# Autodesk Inventor assembly: 200-02-ROCKER-CONNECTOR-ASM-L
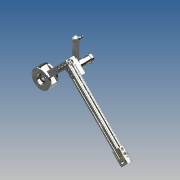
[picture p0: Inventor's stored thumbnail of the model, 180x180]
Saved by Autodesk Inventor 2018.2 (Build 222227000, 227)
## iProperties
Manager: feesmrt
Company: FRANCOR
Created: 2017-12-19
Part Number: 200-02-ROCKER-CONNECTOR-ASM-L
Project: Rescue Robot
Cost Center: -
Material: Generisch
Document SubType Name: Assembly
Designer: feesmrt
Engineer: feesmrt
Authority: feesmrt
Description: Rocker Connector Left Side ASM
Stock Number: 200-02-ROCKER-CONNECTOR-ASM-L
Subject: Rescue Robot
Author: feesmrt
Revision Number: 1
Title: Rocker Connector Left Side ASM
## Documents named in this file (8)
- C:\Users\feesmrt\Documents\FRANC0R\CAD\02-Rocker-Bogie-Robot\200-ROCKER-BOGIE\200-02-ROCKER-CONNECTOR-ASM-L.iam
- C:\Users\feesmrt\Documents\FRANC0R\CAD\02-Rocker-Bogie-Robot\200-ROCKER-BOGIE\200-20-ROCKER-CONNECTOR\200-20-ROCKER-CONNECTOR-ASM-01.iam
- C:\Users\feesmrt\Documents\FRANC0R\CAD\02-Rocker-Bogie-Robot\200-ROCKER-BOGIE\200-30-BOGIE-BEARING\200-30-BOGIE-BEARING-ASM-01.iam
- C:\Users\feesmrt\Documents\FRANC0R\CAD\02-Rocker-Bogie-Robot\200-ROCKER-BOGIE\200-50-WHEEL-CONNECTOR\200-50-WHEEL-CONNECTOR-30MM-ASM-01.iam
- C:\Users\feesmrt\Documents\FRANC0R\CAD\02-Rocker-Bogie-Robot\200-ROCKER-BOGIE\200-20-ROCKER-CONNECTOR\200-20-ROCKER-CONNECTOR-P-01.ipt
- C:\Users\feesmrt\Documents\FRANC0R\CAD\02-Rocker-Bogie-Robot\200-ROCKER-BOGIE\200-20-ROCKER-CONNECTOR\200-20-ROCKER-CONNECTOR-P-02.ipt
- C:\Users\feesmrt\Documents\FRANC0R\CAD\02-Rocker-Bogie-Robot\900-COMPONENTS\900-80-WASHERS\900-80-WASHERS-DIN9021-M8.ipt
- C:\Users\feesmrt\Documents\FRANC0R\CAD\02-Rocker-Bogie-Robot\900-COMPONENTS\900-40-SCREWS\900-40-SCREWS-DIN7984_M8x45.ipt
## Components (15 placed, 7 different names)
1. 200-20-ROCKER-CONNECTOR-ASM-01:1 [sub-assembly] — Passend:1, Fluchtend:1, Fluchtend:2, Fluchtend:3, Passend:3
2. 200-30-BOGIE-BEARING-ASM-01:1 [sub-assembly] — Passend:4, Passend:30, Passend:31
3. 200-50-WHEEL-CONNECTOR-30MM-ASM-01:1 [sub-assembly] — Passend:7, Fluchtend:9, Passend:9
4. 200-20-ROCKER-CONNECTOR-P-01:1 — Passend:1, Fluchtend:1, Fluchtend:2, Passend:2, Passend:4, Passend:30, Passend:31, Passend:10, Passend:11, Passend:14, Passend:15, Passend:18, Passend:19
5. 200-20-ROCKER-CONNECTOR-P-02:1 — Passend:2, Fluchtend:3, Passend:3, Passend:7, Fluchtend:9, Passend:9, Passend:12, Passend:13, Passend:16, Passend:17
6. 900-80-WASHERS-DIN9021-M8:1 — Passend:11, Passend:15, Passend:23, Passend:28
7. 900-80-WASHERS-DIN9021-M8:2 — Passend:10, Passend:14, Passend:22, Passend:27
8. 900-80-WASHERS-DIN9021-M8:3 — Passend:12, Passend:16, Passend:20, Passend:26
9. 900-80-WASHERS-DIN9021-M8:4 — Passend:13, Passend:17, Passend:21, Passend:25
10. 900-80-WASHERS-DIN9021-M8:5 — Passend:18, Passend:19, Passend:24, Passend:29
11. 900-40-SCREWS-DIN7984_M8x45:1 — Passend:22, Passend:27
12. 900-40-SCREWS-DIN7984_M8x45:2 — Passend:23, Passend:28
13. 900-40-SCREWS-DIN7984_M8x45:3 — Passend:24, Passend:29
14. 900-40-SCREWS-DIN7984_M8x45:4 — Passend:20, Passend:26
15. 900-40-SCREWS-DIN7984_M8x45:5 — Passend:21, Passend:25
## Relationships (32: Mate 28, Flush 4)
- Passend:1 [Mate]: 200-20-ROCKER-CONNECTOR-ASM-01:1 ↔ 200-20-ROCKER-CONNECTOR-P-01:1
- Fluchtend:1 [Flush]: 200-20-ROCKER-CONNECTOR-ASM-01:1 ↔ 200-20-ROCKER-CONNECTOR-P-01:1
- Fluchtend:2 [Flush]: 200-20-ROCKER-CONNECTOR-ASM-01:1 ↔ 200-20-ROCKER-CONNECTOR-P-01:1
- Passend:2 [Mate]: 200-20-ROCKER-CONNECTOR-P-01:1 ↔ 200-20-ROCKER-CONNECTOR-P-02:1
- Fluchtend:3 [Flush]: 200-20-ROCKER-CONNECTOR-ASM-01:1 ↔ 200-20-ROCKER-CONNECTOR-P-02:1
- Passend:3 [Mate]: 200-20-ROCKER-CONNECTOR-ASM-01:1 ↔ 200-20-ROCKER-CONNECTOR-P-02:1
- Passend:4 [Mate]: 200-30-BOGIE-BEARING-ASM-01:1 ↔ 200-20-ROCKER-CONNECTOR-P-01:1
- Passend:30 [Mate]: 200-30-BOGIE-BEARING-ASM-01:1 ↔ 200-20-ROCKER-CONNECTOR-P-01:1
- Passend:31 [Mate]: 200-30-BOGIE-BEARING-ASM-01:1 ↔ 200-20-ROCKER-CONNECTOR-P-01:1
- Passend:7 [Mate]: 200-50-WHEEL-CONNECTOR-30MM-ASM-01:1 ↔ 200-20-ROCKER-CONNECTOR-P-02:1
- Fluchtend:9 [Flush]: 200-50-WHEEL-CONNECTOR-30MM-ASM-01:1 ↔ 200-20-ROCKER-CONNECTOR-P-02:1
- Passend:9 [Mate]: 200-50-WHEEL-CONNECTOR-30MM-ASM-01:1 ↔ 200-20-ROCKER-CONNECTOR-P-02:1
- Passend:10 [Mate]: 200-20-ROCKER-CONNECTOR-P-01:1 ↔ 900-80-WASHERS-DIN9021-M8:2
- Passend:11 [Mate]: 200-20-ROCKER-CONNECTOR-P-01:1 ↔ 900-80-WASHERS-DIN9021-M8:1
- Passend:12 [Mate]: 200-20-ROCKER-CONNECTOR-P-02:1 ↔ 900-80-WASHERS-DIN9021-M8:3
- Passend:13 [Mate]: 200-20-ROCKER-CONNECTOR-P-02:1 ↔ 900-80-WASHERS-DIN9021-M8:4
- Passend:14 [Mate]: 200-20-ROCKER-CONNECTOR-P-01:1 ↔ 900-80-WASHERS-DIN9021-M8:2
- Passend:15 [Mate]: 200-20-ROCKER-CONNECTOR-P-01:1 ↔ 900-80-WASHERS-DIN9021-M8:1
- Passend:16 [Mate]: 200-20-ROCKER-CONNECTOR-P-02:1 ↔ 900-80-WASHERS-DIN9021-M8:3
- Passend:17 [Mate]: 200-20-ROCKER-CONNECTOR-P-02:1 ↔ 900-80-WASHERS-DIN9021-M8:4
- Passend:18 [Mate]: 200-20-ROCKER-CONNECTOR-P-01:1 ↔ 900-80-WASHERS-DIN9021-M8:5
- Passend:19 [Mate]: 200-20-ROCKER-CONNECTOR-P-01:1 ↔ 900-80-WASHERS-DIN9021-M8:5
- Passend:20 [Mate]: 900-80-WASHERS-DIN9021-M8:3 ↔ 900-40-SCREWS-DIN7984_M8x45:4
- Passend:21 [Mate]: 900-80-WASHERS-DIN9021-M8:4 ↔ 900-40-SCREWS-DIN7984_M8x45:5
- Passend:22 [Mate]: 900-80-WASHERS-DIN9021-M8:2 ↔ 900-40-SCREWS-DIN7984_M8x45:1
- Passend:23 [Mate]: 900-80-WASHERS-DIN9021-M8:1 ↔ 900-40-SCREWS-DIN7984_M8x45:2
- Passend:24 [Mate]: 900-80-WASHERS-DIN9021-M8:5 ↔ 900-40-SCREWS-DIN7984_M8x45:3
- Passend:25 [Mate]: 900-80-WASHERS-DIN9021-M8:4 ↔ 900-40-SCREWS-DIN7984_M8x45:5
- Passend:26 [Mate]: 900-80-WASHERS-DIN9021-M8:3 ↔ 900-40-SCREWS-DIN7984_M8x45:4
- Passend:27 [Mate]: 900-80-WASHERS-DIN9021-M8:2 ↔ 900-40-SCREWS-DIN7984_M8x45:1
- Passend:28 [Mate]: 900-80-WASHERS-DIN9021-M8:1 ↔ 900-40-SCREWS-DIN7984_M8x45:2
- Passend:29 [Mate]: 900-80-WASHERS-DIN9021-M8:5 ↔ 900-40-SCREWS-DIN7984_M8x45:3
